# Autodesk Inventor assembly: hexapod_v0.1
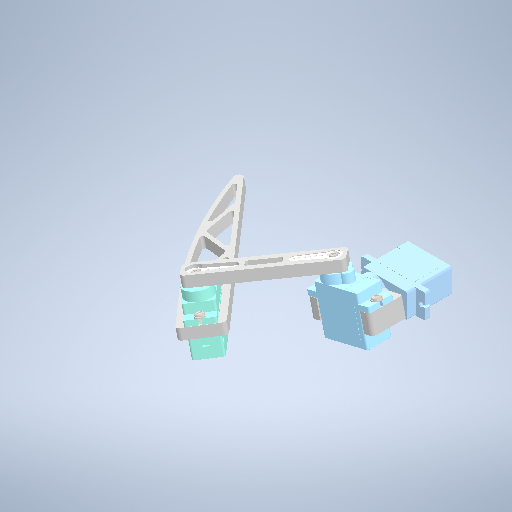
[picture p0: Inventor's stored thumbnail of the model, 512x512]
Saved by Autodesk Inventor 2025 (Build 290162000, 162)
## iProperties
Created: 2024-06-04
Part Number: hexapod_v0.1
Document SubType Name: Assembly
Designer: sgols
Author: sgols
## Documents named in this file (8)
- C:\git\hexapod\mechanics\Leg Left v0.1.iam
- C:\git\hexapod\mechanics\Servos\Micro Servo 9g\SG90 - Micro Servo 9g - Tower Pro.1\SG90 - Micro Servo 9g - Tower Pro.1.ipt
- C:\git\hexapod\mechanics\Servos\Micro Servo 9g\SG90 - Micro Servo 9g - Tower Pro.2\SG90 - Micro Servo 9g - Tower Pro.2.ipt
- C:\git\hexapod\mechanics\Servos\Micro Servo 9g\SG90 - Micro Servo 9g - Tower Pro.5\SG90 - Micro Servo 9g - Tower Pro.5.ipt
- C:\git\hexapod\mechanics\Servos\Micro Servo 9g\SG90 - Micro Servo 9g - Tower Pro.6\SG90 - Micro Servo 9g - Tower Pro.6.ipt
- C:\git\hexapod\mechanics\Hip v0.1.ipt
- C:\git\hexapod\mechanics\Femur v0.1.ipt
- C:\git\hexapod\mechanics\Foot v0.1.ipt
## Components (16 placed, 9 different names)
1. Femur v0.1:1 — Insert:1, Mate:1, Insert:10, Mate:11
2. Foot v0.1:1 — Mate:5, Mate:16, Angle:1
3. Hip v0.1:1 — Mate:9, Mate:14, Mate:10, Mate:15, Mate:17, Angle:2
4. SG90 - Micro Servo 9g - Tower Pro.6:3 — Insert:9
5. SG90 - Micro Servo 9g - Tower Pro.5:4 — Insert:7
6. SG90 - Micro Servo 9g - Tower Pro.5:3 — Insert:6
7. SG90 - Micro Servo 9g - Tower Pro.6:2 — Insert:5
8. SG90 - Micro Servo 9g - Tower Pro.6:1 — Insert:4
9. SG90 - Micro Servo 9g - Tower Pro.5:2 — Insert:3
10. SG90 - Micro Servo 9g - Tower Pro.5:1 — Insert:2
11. Servo Hip — Rotational:3, Mate:12, Mate:13, Flush:1
12. Servo Femur — Rotational:2, Mate:9, Insert:6, Insert:7, Mate:17, Angle:2
13. Servo Foot — Mate:5, Insert:2, Insert:3, Rotational:1, Mate:16, Angle:1
14. SG90 - Micro Servo 9g - Tower Pro.2:2 — Rotational:2, Insert:5, Insert:10, Mate:11
15. SG90 - Micro Servo 9g - Tower Pro.2:1 — Insert:1, Mate:1, Rotational:1, Insert:4
16. SG90 - Micro Servo 9g - Tower Pro.2:3 — Mate:14, Mate:10, Insert:9, Rotational:3, Mate:15
## Relationships (26: Mate 11, Insert 9, RevoluteJoint 3, Angle 2, Flush 1)
- Insert:1: Femur v0.1:1 ↔ SG90 - Micro Servo 9g - Tower Pro.2:1
- Mate:1: Femur v0.1:1 ↔ SG90 - Micro Servo 9g - Tower Pro.2:1
- Mate:5: Foot v0.1:1 ↔ Servo Foot
- Insert:2: SG90 - Micro Servo 9g - Tower Pro.5:1 ↔ Servo Foot
- Insert:3: SG90 - Micro Servo 9g - Tower Pro.5:2 ↔ Servo Foot
- Rotational:1 [RevoluteJoint]: Servo Foot ↔ SG90 - Micro Servo 9g - Tower Pro.2:1
- Insert:4: SG90 - Micro Servo 9g - Tower Pro.6:1 ↔ SG90 - Micro Servo 9g - Tower Pro.2:1
- Rotational:2 [RevoluteJoint]: Servo Femur ↔ SG90 - Micro Servo 9g - Tower Pro.2:2
- Insert:5: SG90 - Micro Servo 9g - Tower Pro.6:2 ↔ SG90 - Micro Servo 9g - Tower Pro.2:2
- Mate:9: Hip v0.1:1 ↔ Servo Femur
- Insert:6: SG90 - Micro Servo 9g - Tower Pro.5:3 ↔ Servo Femur
- Insert:7: SG90 - Micro Servo 9g - Tower Pro.5:4 ↔ Servo Femur
- Mate:14: Hip v0.1:1 ↔ SG90 - Micro Servo 9g - Tower Pro.2:3
- Mate:10: Hip v0.1:1 ↔ SG90 - Micro Servo 9g - Tower Pro.2:3
- Insert:9: SG90 - Micro Servo 9g - Tower Pro.6:3 ↔ SG90 - Micro Servo 9g - Tower Pro.2:3
- Insert:10: Femur v0.1:1 ↔ SG90 - Micro Servo 9g - Tower Pro.2:2
- Mate:11: Femur v0.1:1 ↔ SG90 - Micro Servo 9g - Tower Pro.2:2
- Rotational:3 [RevoluteJoint]: Servo Hip ↔ SG90 - Micro Servo 9g - Tower Pro.2:3
- Mate:12: Servo Hip
- Mate:13: Servo Hip
- Flush:1: Servo Hip
- Mate:15: Hip v0.1:1 ↔ SG90 - Micro Servo 9g - Tower Pro.2:3
- Mate:16: Foot v0.1:1 ↔ Servo Foot
- Mate:17: Hip v0.1:1 ↔ Servo Femur
- Angle:1 (0 deg): Foot v0.1:1 ↔ Servo Foot
- Angle:2 (0 deg): Hip v0.1:1 ↔ Servo Femur
